# Autodesk Inventor assembly: Wheel Assembly
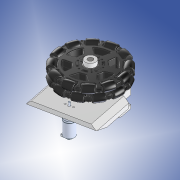
[picture p0: Inventor's stored thumbnail of the model, 180x180]
Saved by Autodesk Inventor 2017 SP1 (Build 210196100, 196)
## iProperties
Created: 2017-08-01
Part Number: Wheel Assembly
Document SubType Name: Assembly
Designer: Zach
Author: Zach
## Documents named in this file (8)
- C:\Users\Zach\Documents\GitHub\cr-laundry-robot\src\Base 2\Wheel Assembly\Wheel Assembly.iam
- C:\Users\Zach\Documents\GitHub\cr-laundry-robot\src\Base 2\Wheel Assembly\WA001.ipt
- C:\Users\Zach\Documents\GitHub\cr-laundry-robot\lib\Omni Wheel 6in\217-2585.ipt
- C:\Users\Zach\Documents\GitHub\cr-laundry-robot\lib\28x12x8mm Bearing.ipt
- C:\Users\Zach\Documents\GitHub\cr-laundry-robot\src\Base 2\Wheel Assembly\WA002.ipt
- C:\Users\Zach\Documents\GitHub\cr-laundry-robot\src\Base 2\Wheel Assembly\WA003.ip.ipt
- C:\Users\Zach\Documents\GitHub\cr-laundry-robot\src\Base 2\Wheel Assembly\WA004.ipt
- C:\Users\Zach\Documents\GitHub\cr-laundry-robot\lib\DC Motor with Encoder\Motor.ipt
## Components (10 placed, 7 different names)
1. WA001:1 — Mate:3, Mate:7, Flush:3, Mate:9, Mate:10, Mate:11
2. 217-2585:1 — Mate:1, Flush:1, Mate:2, Flush:2, Mate:5, Mate:6, Mate:8
3. 28x12x8mm Bearing:1 — Mate:1, Flush:1, Mate:3, Mate:4
4. 28x12x8mm Bearing:2 — Mate:2, Flush:2
5. WA002:1 — Mate:4, Mate:5, Mate:6, Mate:12, Mate:13
6. WA003.ip:1 — Mate:7, Mate:8, Flush:3
7. WA004:1 — Mate:9, Mate:13, Mate:14, Mate:15, Mate:16, Mate:17, Mate:18, Mate:19, Mate:20
8. Motor:1 — Mate:14, Mate:15, Mate:16
9. 28x12x8mm Bearing:3 — Mate:19, Mate:20
10. 28x12x8mm Bearing:4 — Mate:17, Mate:18
## Relationships (23: Mate 20, Flush 3)
- Mate:1: 217-2585:1 ↔ 28x12x8mm Bearing:1
- Flush:1: 217-2585:1 ↔ 28x12x8mm Bearing:1
- Mate:2: 217-2585:1 ↔ 28x12x8mm Bearing:2
- Flush:2: 217-2585:1 ↔ 28x12x8mm Bearing:2
- Mate:3: WA001:1 ↔ 28x12x8mm Bearing:1
- Mate:4: 28x12x8mm Bearing:1 ↔ WA002:1
- Mate:5: 217-2585:1 ↔ WA002:1
- Mate:6: 217-2585:1 ↔ WA002:1
- Mate:7: WA001:1 ↔ WA003.ip:1
- Mate:8: 217-2585:1 ↔ WA003.ip:1
- Flush:3: WA001:1 ↔ WA003.ip:1
- Mate:9: WA001:1 ↔ WA004:1
- Mate:10: WA001:1
- Mate:11: WA001:1
- Mate:12: WA002:1
- Mate:13: WA002:1 ↔ WA004:1
- Mate:14: WA004:1 ↔ Motor:1
- Mate:15: WA004:1 ↔ Motor:1
- Mate:16: WA004:1 ↔ Motor:1
- Mate:17: WA004:1 ↔ 28x12x8mm Bearing:4
- Mate:18: WA004:1 ↔ 28x12x8mm Bearing:4
- Mate:19: WA004:1 ↔ 28x12x8mm Bearing:3
- Mate:20: WA004:1 ↔ 28x12x8mm Bearing:3
